# Autodesk Inventor assembly: Stapler
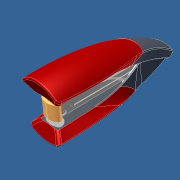
[picture p0: Inventor's stored thumbnail of the model, 180x180]
Saved by Autodesk Inventor 2011 (Build 150239000, 239)
## iProperties
Shininess: 64.0
Length Units: 11272
Angle Units: 11279
Time Units: 11290
Mass Units: 11286
Length Display Precision: 3
Angle Display Precision: 2
Compacted: True
Part Number: Stapler
Document SubType Name: Assembly
Created: 2002-09-25
Designer: Autodesk, Inc.
Project: Inventor Samples
Mass: 654.978 g
Surface Area: 878.347 cm^2
Volume: 123.25 cm^3
Density: 5.31422 g/cm^3
Density: 0.0
Volumn: 0.0
Area: 0.0
PropertySet Name: Model Information
Control State: 0
Master: False
Checked Out: False
Subject: Inventor Samples
Author: Autodesk, Inc.
Revision Number: A
## Documents named in this file (3)
- C:\Users\Public\Documents\Autodesk\Inventor 2011\Samples\Models\Assemblies\Stapler\Stapler.iam
- C:\Users\Public\Documents\Autodesk\Inventor 2011\Samples\Models\Assemblies\Stapler\Components\Bottom.iam
- C:\Users\Public\Documents\Autodesk\Inventor 2011\Samples\Models\Assemblies\Stapler\Components\Upper.iam
## Components (2 placed, 2 different names)
1. Bottom:1 [sub-assembly] — Flush:1, Mate:1
2. Upper:1 [sub-assembly] — Flush:1, Mate:1, Angle:1
## Relationships (3: Flush 1, Mate 1, Angle 1)
- Flush:1: Bottom:1 ↔ Upper:1
- Mate:1: Bottom:1 ↔ Upper:1
- Angle:1 (180 deg): Upper:1
